# Autodesk Inventor assembly: Lidar Sensor Lexan Assembly
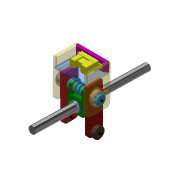
[picture p0: Inventor's stored thumbnail of the model, 180x180]
Saved by Autodesk Inventor 2018.3 (Build 223284000, 284)
## iProperties
Created: 2019-02-26
Part Number: Lidar Sensor Lexan Assembly
Document SubType Name: Assembly
Designer: aye06091
Mass: 149.971 g
Surface Area: 692.089 cm^2
Volume: 122.791 cm^3
Density: 1.22135 g/cm^3
Author: aye06091
## Documents named in this file (17)
- Y:\DeSimony-R\Senior R&D\4 R&D Shared Folder\VisiStick\VisiStick (Inventor)\Case Final - Version 4\Lidar Sensor Lexan Assembly.iam
- Y:\DeSimony-R\Senior R&D\4 R&D Shared Folder\VisiStick\VisiStick (Inventor)\Case Final - Version 4\Lidar Sensor Case Piece 3.ipt
- Y:\DeSimony-R\Senior R&D\4 R&D Shared Folder\VisiStick\VisiStick (Inventor)\Electronics\Sharp 2Y0A02.ipt
- Y:\DeSimony-R\Senior R&D\4 R&D Shared Folder\VisiStick\VisiStick (Inventor)\Physical Parts\Lidar Sensor Case 4 v2.ipt
- Y:\DeSimony-R\Senior R&D\4 R&D Shared Folder\VisiStick\VisiStick (Inventor)\Case Final - Version 4\Ball Bearing.ipt
- Y:\DeSimony-R\Senior R&D\4 R&D Shared Folder\VisiStick\VisiStick (Inventor)\Case Final - Version 4\Steel Rod.ipt
- Y:\DeSimony-R\Senior R&D\4 R&D Shared Folder\VisiStick\VisiStick (Inventor)\Physical Parts\T-Spacer .125 inch bore.ipt
- Y:\DeSimony-R\Senior R&D\4 R&D Shared Folder\VisiStick\VisiStick (Inventor)\Physical Parts\Cane Segmant.ipt
- Y:\DeSimony-R\Senior R&D\4 R&D Shared Folder\VisiStick\VisiStick (Inventor)\Case Final - Version 4\Smaller Needle Bearing Mount.ipt
- Y:\DeSimony-R\Senior R&D\4 R&D Shared Folder\VisiStick\VisiStick (Inventor)\Physical Parts\Lidar Sensor Case v4 Piece 1.ipt
- Y:\DeSimony-R\Senior R&D\4 R&D Shared Folder\VisiStick\VisiStick (Inventor)\Physical Parts\Lidar Sensor Case v4 Piece 2.ipt
- Y:\DeSimony-R\Senior R&D\4 R&D Shared Folder\VisiStick\VisiStick (Inventor)\Physical Parts\Lidar Sensor Case v4 Piece 3.ipt
- Y:\DeSimony-R\Senior R&D\4 R&D Shared Folder\VisiStick\VisiStick (Inventor)\Physical Parts\Bronze.ipt
- Y:\DeSimony-R\Senior R&D\4 R&D Shared Folder\VisiStick\VisiStick (Inventor)\Physical Parts\.5in Bore Needle Bearing.ipt
- Y:\DeSimony-R\Senior R&D\4 R&D Shared Folder\VisiStick\VisiStick (Inventor)\Physical Parts\.02in Washer.ipt
- Y:\DeSimony-R\Senior R&D\4 R&D Shared Folder\VisiStick\VisiStick (Inventor)\Physical Parts\1in Rod.ipt
- Y:\DeSimony-R\Senior R&D\4 R&D Shared Folder\VisiStick\VisiStick (Inventor)\Physical Parts\Needle Bearing Stopper.ipt
## Components (30 placed, 16 different names)
1. Sharp 2Y0A02:1 — Insert:5, Insert:6
2. Ball Bearing:1 — Insert:18, Insert:25, Insert:33
3. Ball Bearing:2 — Insert:19, Insert:26, Insert:32
4. Steel Rod:1 — Mate:6, Mate:13, Mate:16, Mate:24
5. Lidar Sensor Case 4 v2:1 — Mate:18, Mate:19, Flush:2
6. Lidar Sensor Case Piece 3:1 — Insert:5, Insert:6, Mate:20, Flush:4, Mate:21, Mate:22, Flush:6
7. T-Spacer .125 inch bore:1 — Insert:16
8. T-Spacer .125 inch bore:2 — Insert:18
9. T-Spacer .125 inch bore:3 — Insert:19, Mate:24, Mate:25
10. T-Spacer .125 inch bore:4 — Insert:16, Insert:17
11. T-Spacer .125 inch bore:5 — Insert:17, Insert:23
12. Cane Segmant:1 — Insert:29
13. Smaller Needle Bearing Mount:1 — Mate:6, Mate:13, Insert:22, Mate:25, Insert:28, Insert:30, Insert:31, Insert:34
14. T-Spacer .125 inch bore:6 — Insert:22, Insert:23
15. Lidar Sensor Case v4 Piece 1:1 — Insert:25, Mate:17, Tangent:2, Flush:5, Flush:7, Insert:37, Insert:40
16. Lidar Sensor Case v4 Piece 1:2 — Insert:26, Flush:5, Mate:23, Flush:7, Insert:38, Insert:39
17. Lidar Sensor Case v4 Piece 2:1 — Mate:16, Mate:17, Tangent:2, Flush:1, Mate:18, Flush:2, Mate:21, Mate:22, Flush:6
18. Lidar Sensor Case v4 Piece 3:1 — Flush:1, Mate:19, Mate:20, Flush:4, Mate:23
19. Bronze:1 — Insert:37
20. Bronze:2 — Insert:38
21. .5in Bore Needle Bearing:1 — Insert:28, Insert:29, Insert:41, Insert:42
22. T-Spacer .125 inch bore:7 — Insert:30
23. T-Spacer .125 inch bore:8 — Insert:31
24. T-Spacer .125 inch bore:9 — Insert:32
25. T-Spacer .125 inch bore:10 — Insert:33
26. .02in Washer:1 — Insert:34
27. 1in Rod:1 — Insert:40
28. 1in Rod:2 — Insert:39
29. Needle Bearing Stopper:1 — Insert:42
30. Needle Bearing Stopper:2 — Insert:41
## Relationships (42: Insert 23, Mate 12, Flush 6, Tangent 1)
- Insert:5: Sharp 2Y0A02:1 ↔ Lidar Sensor Case Piece 3:1
- Insert:6: Sharp 2Y0A02:1 ↔ Lidar Sensor Case Piece 3:1
- Insert:16: T-Spacer .125 inch bore:1 ↔ T-Spacer .125 inch bore:4
- Insert:17: T-Spacer .125 inch bore:4 ↔ T-Spacer .125 inch bore:5
- Mate:6: Steel Rod:1 ↔ Smaller Needle Bearing Mount:1
- Insert:18: Ball Bearing:1 ↔ T-Spacer .125 inch bore:2
- Insert:19: Ball Bearing:2 ↔ T-Spacer .125 inch bore:3
- Mate:13: Steel Rod:1 ↔ Smaller Needle Bearing Mount:1
- Insert:22: Smaller Needle Bearing Mount:1 ↔ T-Spacer .125 inch bore:6
- Insert:23: T-Spacer .125 inch bore:5 ↔ T-Spacer .125 inch bore:6
- Insert:25: Ball Bearing:1 ↔ Lidar Sensor Case v4 Piece 1:1
- Insert:26: Ball Bearing:2 ↔ Lidar Sensor Case v4 Piece 1:2
- Mate:16: Steel Rod:1 ↔ Lidar Sensor Case v4 Piece 2:1
- Mate:17: Lidar Sensor Case v4 Piece 1:1 ↔ Lidar Sensor Case v4 Piece 2:1
- Tangent:2: Lidar Sensor Case v4 Piece 1:1 ↔ Lidar Sensor Case v4 Piece 2:1
- Flush:1: Lidar Sensor Case v4 Piece 2:1 ↔ Lidar Sensor Case v4 Piece 3:1
- Mate:18: Lidar Sensor Case 4 v2:1 ↔ Lidar Sensor Case v4 Piece 2:1
- Mate:19: Lidar Sensor Case 4 v2:1 ↔ Lidar Sensor Case v4 Piece 3:1
- Flush:2: Lidar Sensor Case 4 v2:1 ↔ Lidar Sensor Case v4 Piece 2:1
- Mate:20: Lidar Sensor Case Piece 3:1 ↔ Lidar Sensor Case v4 Piece 3:1
- Flush:4: Lidar Sensor Case Piece 3:1 ↔ Lidar Sensor Case v4 Piece 3:1
- Flush:5: Lidar Sensor Case v4 Piece 1:1 ↔ Lidar Sensor Case v4 Piece 1:2
- Mate:21: Lidar Sensor Case Piece 3:1 ↔ Lidar Sensor Case v4 Piece 2:1
- Mate:22: Lidar Sensor Case Piece 3:1 ↔ Lidar Sensor Case v4 Piece 2:1
- Flush:6: Lidar Sensor Case Piece 3:1 ↔ Lidar Sensor Case v4 Piece 2:1
- Mate:23: Lidar Sensor Case v4 Piece 1:2 ↔ Lidar Sensor Case v4 Piece 3:1
- Flush:7: Lidar Sensor Case v4 Piece 1:1 ↔ Lidar Sensor Case v4 Piece 1:2
- Mate:24: Steel Rod:1 ↔ T-Spacer .125 inch bore:3
- Mate:25 (2.3707 mm): T-Spacer .125 inch bore:3 ↔ Smaller Needle Bearing Mount:1
- Insert:28 (-1.5875 mm): Smaller Needle Bearing Mount:1 ↔ .5in Bore Needle Bearing:1
- Insert:29 (-76.2 mm): Cane Segmant:1 ↔ .5in Bore Needle Bearing:1
- Insert:30: Smaller Needle Bearing Mount:1 ↔ T-Spacer .125 inch bore:7
- Insert:31: Smaller Needle Bearing Mount:1 ↔ T-Spacer .125 inch bore:8
- Insert:32: Ball Bearing:2 ↔ T-Spacer .125 inch bore:9
- Insert:33: Ball Bearing:1 ↔ T-Spacer .125 inch bore:10
- Insert:34: Smaller Needle Bearing Mount:1 ↔ .02in Washer:1
- Insert:37: Lidar Sensor Case v4 Piece 1:1 ↔ Bronze:1
- Insert:38: Lidar Sensor Case v4 Piece 1:2 ↔ Bronze:2
- Insert:39 (-10.795 mm): Lidar Sensor Case v4 Piece 1:2 ↔ 1in Rod:2
- Insert:40 (-10.795 mm): Lidar Sensor Case v4 Piece 1:1 ↔ 1in Rod:1
- Insert:41: .5in Bore Needle Bearing:1 ↔ Needle Bearing Stopper:2
- Insert:42: .5in Bore Needle Bearing:1 ↔ Needle Bearing Stopper:1
